# Autodesk Inventor assembly: Single Acting Piston
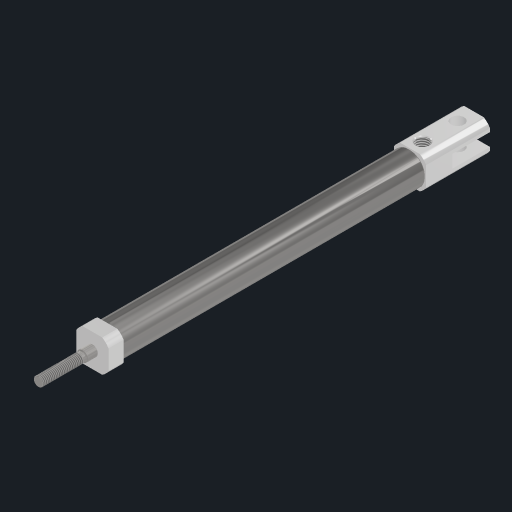
[picture p0: Inventor's stored thumbnail of the model, 512x512]
Saved by Autodesk Inventor 2023 (Build 270158030, 158C)
## iProperties
Created: 2022-09-23
Part Number: Single Acting Piston
Document SubType Name: Assembly
Designer: maxxw
Mass: 12.2112 g
Surface Area: 100.21 cm^2
Volume: 12.2112 cm^3
Density: 1 g/cm^3
Author: maxxw
## Documents named in this file (3)
- C:\Users\maxxw\Documents\GitHub\VEX-CAD-Inventor\Motion\Pneumatics\Single Acting Piston.iam
- C:\Users\maxxw\Documents\GitHub\VEX-CAD-Inventor\Motion\Pneumatics\Reference Parts\Pistons\Single Acting Piston Rod.ipt
- C:\Users\maxxw\Documents\GitHub\VEX-CAD-Inventor\Motion\Pneumatics\Reference Parts\Pistons\Single Acting Piston Body.ipt
## Components (2 placed, 2 different names)
1. Single Acting Piston Rod:1 — Mate:1, Mate:2
2. Single Acting Piston Body:1 — Mate:1, Mate:2
## Relationships (2: Mate 2)
- Mate:1: Single Acting Piston Rod:1 ↔ Single Acting Piston Body:1
- Mate:2: Single Acting Piston Rod:1 ↔ Single Acting Piston Body:1
